# Autodesk Inventor assembly: Lower Goal
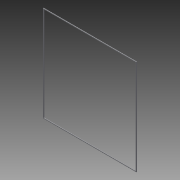
[picture p0: Inventor's stored thumbnail of the model, 180x180]
Saved by Autodesk Inventor 2014 (Build 180170000, 170)
## iProperties
Created: 2014-01-29
Part Number: Lower Goal
Document SubType Name: Assembly
Designer: NilesStanton
Author: NilesStanton
## Documents named in this file (3)
- C:\GitHub\team3566-2014\CAD\Court\Lower Goal.iam
- C:\GitHub\team3566-2014\CAD\Court\Lower Goal Longer.ipt
- C:\GitHub\team3566-2014\CAD\Court\Part4.ipt
## Components (4 placed, 2 different names)
1. Lower Goal Longer:1 — Flush:1, Flush:2, Flush:3, Flush:4, Flush:5, Flush:6
2. Lower Goal Longer:2 — Flush:7, Flush:8, Flush:9
3. Part4:1 — Flush:4, Flush:5, Flush:6
4. Part4:2 — Flush:1, Flush:2, Flush:3, Flush:7, Flush:8, Flush:9
## Relationships (9: Flush 9)
- Flush:1: Lower Goal Longer:1 ↔ Part4:2
- Flush:2: Lower Goal Longer:1 ↔ Part4:2
- Flush:3: Lower Goal Longer:1 ↔ Part4:2
- Flush:4: Lower Goal Longer:1 ↔ Part4:1
- Flush:5: Lower Goal Longer:1 ↔ Part4:1
- Flush:6: Lower Goal Longer:1 ↔ Part4:1
- Flush:7: Lower Goal Longer:2 ↔ Part4:2
- Flush:8: Lower Goal Longer:2 ↔ Part4:2
- Flush:9: Lower Goal Longer:2 ↔ Part4:2
